# Autodesk Inventor assembly: KZBN17-113-P14-LA25-TC4-TB4-KB21-HB50-ZA3-HA18-AA120
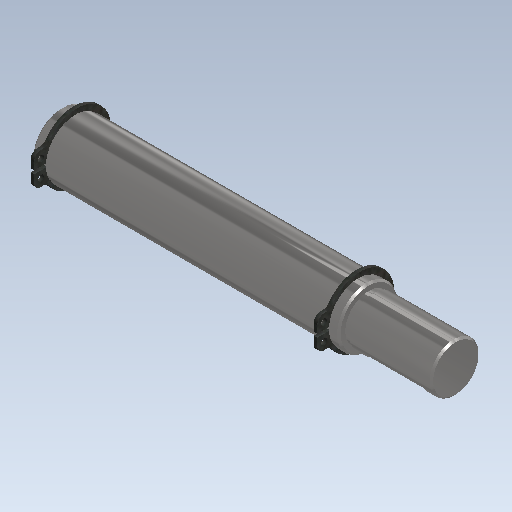
[picture p0: Inventor's stored thumbnail of the model, 512x512]
Saved by Autodesk Inventor 2021.3 (Build 253353000, 353)
## iProperties
Part Number: KZBN17-113-P14-LA25-TC4-TB4-KB21-HB50-ZA3-HA18-AA120
Catalog Web Link: www.cadenas.de
Description: KZBE, KZBN, KZBC, KZBP, KZBF-Driving Shaft - One End Stepped -
Vendor: MISUMI
Document SubType Name: Assembly
Designer: partserver
Manufacturer: MISUMI
Mass: 22.9238 g
Surface Area: 74.0466 cm^2
Volume: 22.9238 cm^3
Density: 1 g/cm^3
Category: PARTsolutions
Company: MISUMI
PSOL_IDENT_0: {$CADENAS_DATA\23d-libs\misumi\metric\11_rotary_shafts\kzbc_asmtab.prj},748 {VTYP=3D},{STYP=ASSTAB},
PSOL_IDENT_1: {NB=KZBN17-113-P14-LA25-TC4-TB4-KB21-HB50-ZA3-HA18-AA120},{LINA=KZBN17-113-P14-LA25-TC4-TB4-KB21-HB5
PSOL_IDENT_2: 0-ZA3-HA18-AA120},{NN=KZBE, KZBN, KZBC, KZBP, KZBF},{DATE=27.07.2021 05:05:24},{GEOMDATE=01.11.2019
PSOL_IDENT_3: 08:16:05},{VERSION=},{LINEID=60},{WBVAR=TS,HARD,ST,L,P,LA,ALT1,MA,MSA,MMA,ALT4,MD,MSD,MMD,ALT2,MB,MS
PSOL_IDENT_4: B,MMB,ALT5,NA,NBALT5,ALT7,TA,ALT6,TC,TB,ALT9,KA,HAALT9,ALT10,KB,HBALT10,KC,HCALT10,ALT12,ZA,HAALT12,
PSOL_IDENT_5: AAALT12,ALT13,ZB,HBALT13,ABALT13,ZC,HCALT13,ACALT13,ALT15,SA,ALT16,SC,ALT18,WA,GA,AAALT18,ALT19,WB,G
PSOL_IDENT_6: B,ABALT19,WC,GC,ACALT19},{WBNUMERIC=L,P,LA,MA,MSA,MMA,MD,MSD,MMD,MB,MSB,MMB,TA,TC,TB,KA,HAALT9,KB,HB
PSOL_IDENT_7: ALT10,KC,HCALT10,ZA,HAALT12,AAALT12,ZB,HBALT13,ABALT13,ZC,HCALT13,ACALT13,SA,SC,WA,GA,AAALT18,WB,GB,
PSOL_IDENT_8: ABALT19,WC,GC,ACALT19}  {NB=KZBN17-113-P14-LA25-TC4-TB4-KB21-HB50-ZA3-HA18-AA120},{LINA=KZBN17-113-P
PSOL_IDENT_9: 14-LA25-TC4-TB4-KB21-HB50-ZA3-HA18-AA120},{KT=DUMMY},{PN=KZBN17-113-P14-LA25-TC4-TB4-KB21-HB50-ZA3-H
PSOL_IDENT_10: A18-AA120},{TYPE=KZBN},{D=17},{TS=h6},{TSALG= 'h7','h7','h6','h6' },{HARD=-},{HARDALG= '-','-','IHSH
PSOL_IDENT_11: 50','Induction Hardened Surface Hardness 50HRC' },{ST=-},{STALG= '-','-','BO','Black Oxide','ENP','E
PSOL_IDENT_12: lectroless Nickel Plating'},{L=113.0},{LALG=[100:400/0.5]},{P=14},{PALG=[10:16/1]},{PMIN=10},{PMAX=1
PSOL_IDENT_13: 6},{LA=25.0},{LAALG=[10:56.5/0.5]},{LAMIN=10.0},{LAMAX=56.5},{CIFCC=0.5},{CIFR=0.0},{ALT1=},{ALT1ALG=
PSOL_IDENT_14: '','Not applicable' },{ALT1PN=},{MA=0},{MAALG=[0]},{MAMIN=0},{MAMAX=0},{MSA=0},{MSAALG=[0]},{MSAMIN=
PSOL_IDENT_15: 0},{MSAMAX=0},{MMA=0},{MMAALG=[0]},{MMAMIN=0},{MMAMAX=0},{MALT1=0},{APITCH=0.00},{ALT4=},{ALT4ALG= ''
PSOL_IDENT_16: ,'w/o Shaft End D Threaded Left End','MSD','with MSD (Fine (Standard) JIS 6h (Class 2))','MMD','with
PSOL_IDENT_17: MMD (Fine (Precision) JIS 4h (Class 1))' },{ALT4PN=},{MD=0},{MDALG=[0]},{MDMIN=0},{MDMAX=0},{MSD=0}
PSOL_IDENT_18: ,{MSDALG=[0]},{MSDMIN=0},{MSDMAX=0},{MMD=0},{MMDALG=[0]},{MMDMIN=0},{MMDMAX=0},{MALT4=0},{DPITCH=0.0
PSOL_IDENT_19: 0},{MDPITCH=0},{MSDPITCH=1},{ALT2=},{ALT2ALG= '','w/o Shaft End D Threaded Right End','MSB','with MS
PSOL_IDENT_20: B (Fine (Standard) JIS 6h (Class 2))','MMB','with MMB (Fine (Precision) JIS 4h (Class 1))' },{ALT2PN=
PSOL_IDENT_21: },{MB=0},{MBALG=[0]},{MBMIN=0},{MBMAX=0},{MSB=0},{MSBALG=[0]},{MSBMIN=0},{MSBMAX=0},{MMB=0},{MMBALG=
PSOL_IDENT_22: [0]},{MMBMIN=0},{MMBMAX=0},{MALT2=0},{BPITCH=0.00},{ALT5=},{ALT5ALG= '','w/o Tapped Ends','NA','with
PSOL_IDENT_23: NA (Tapped Left End)','NB','with NB (Tapped Right End)','NANB','with NA + NB (Tapped Both Ends)' },
PSOL_IDENT_24: {ALT5PN=},{NA=0},{NAALG= '0','N/A' },{NAMAX=10},{NA1=0},{NAL=0},{PITCHA=0},{NBALT5=0},{NBALT5ALG= '0'
PSOL_IDENT_25: ,'N/A' },{NBMAX=12},{NBMAX1=24},{NBMAX2=12},{NBMAX3=12},{NBMAX4=0},{NB1=0},{NBL=0},{PITCHB=0},{CIFNA=
PSOL_IDENT_26: 0},{ALT7=},{ALT7ALG=  '','w/o Shaft End P Retaining Ring Groove','TA','with TA (Shaft End P Retainin
PSOL_IDENT_27: g Ring Groove)' },{ALT7PN=},{TA=0},{TAALG=[0]},{TAMIN=4},{TAMAX=22},{DDALT7=0.0},{MMALT7=0.00},{ALT6=
PSOL_IDENT_28: TCTB},{ALT6ALG=  '','w/o Shaft End D Retaining Ring Grooves','TC','with TC (Shaft End D Retaining Ri
PSOL_IDENT_29: ng Groove Left End)','TB','with TB (Shaft End D Retaining Ring Groove Right End)','TCTB','with TC +
PSOL_IDENT_30: TB (Shaft End D Retaining Ring Grooves Both Ends)' },{ALT6PN=-TC4-TB4},{TC=4},{TCALG=[4:82/1]},{TCMI
PSOL_IDENT_31: N=4},{TCMAX=82},{TB=4},{TBALG=[4:86/1]},{TBMIN=4},{TBMAX=86},{DDALT6=16.2},{MMALT6=1.15},{ALT9=},{AL
PSOL_IDENT_32: T9ALG= '','w/o Shaft End P Key Groove','KA','with KA (Shaft End P Key Groove)' },{ALT9PN=},{KA=0},{K
PSOL_IDENT_33: AALG=[0]},{KAMIN=0},{KAMAX=18},{HAALT9=0},{HAALT9ALG=[0]},{HAALT9MIN=5},{HAALT9MAX=23},{PBB=5},{PTT=
PSOL_IDENT_34: 3.0},{ALT10=KB},{ALT10ALG= '','w/o Shaft End D Key Grooves','KB','with KB (Shaft End D Key Groove)','
PSOL_IDENT_35: KBKC','with KB + KC (Shaft End D Two Key Grooves)' },{ALT10PN=-KB21-HB50},{KB=21},{KBALG=[2:83/1]},{
PSOL_IDENT_36: KBMIN=2},{KBMAX1=83},{KBMAX2=76},{HBALT10=50},{HBALT10ALG=[5:67/1]},{HBALT10MIN=5},{HBALT10MAX1=67},
PSOL_IDENT_37: {HBALT10MAX2=60},{KC=0},{KCALG=[0]},{KCMIN=73},{KCMAX=83},{HCALT10=0},{HCALT10ALG=[0]},{HCALT10MIN=5
PSOL_IDENT_38: },{HCALT10MAX=88},{DBB=5},{DTT=3.0},{ALT12=ZA},{ALT12ALG= '','w/o Shaft End P Key Groove + Set Screw
PSOL_IDENT_39: Flat','ZA','with ZA (Shaft End P Key Groove + Set Screw Flat)' },{ALT12PN=-ZA3-HA18-AA120},{ZA=3},{
PSOL_IDENT_40: ZAALG=[0:18/1]},{ZAMIN=0},{ZAMAX=18},{HAALT12=18},{HAALT12ALG=[5:20/1]},{HAALT12MIN=5},{HAALT12MAX=2
PSOL_IDENT_41: 0},{AAALT12=120},{AAALT12ALG=[60:300/30]},{PH=1},{ALT13=},{ALT13ALG= '','Not applicable' },{ALT13PN=
PSOL_IDENT_42: },{ZB=0},{ZBALG=[0]},{ZBMIN=2},{ZBMAX1=83},{ZBMAX2=76},{HBALT13=0},{HBALT13ALG=[0]},{HBALT13MIN=5},{
PSOL_IDENT_43: HBALT13MAX1=88},{HBALT13MAX2=81},{ABALT13=0},{ABALT13ALG=[0]},{ZC=0},{ZCALG=[0]},{ZCMIN=2},{ZCMAX=83
PSOL_IDENT_44: },{HCALT13=0},{HCALT13ALG=[0]},{HCALT13MIN=5},{HCALT13MAX=88},{ACALT13=0},{ACALT13ALG=[0]},{DH=0},{A
PSOL_IDENT_45: LT15=},{ALT15ALG= '', 'w/o Shaft End P Wrench Flats', 'SA', 'with SA (Shaft End P Wrench Flats)' },{
PSOL_IDENT_46: ALT15PN=},{SA=0},{SAALG=[0]},{SAMIN=0},{SAMAX=25},{WALT15=0.0},{LLALT15=0},{ALT16=},{ALT16ALG= '', '
PSOL_IDENT_47: w/o Shaft End D Wrench Flats', 'SC', 'with SC (Shaft End D Wrench Flats)' },{ALT16PN=},{SC=0},{SCALG=
PSOL_IDENT_48: [0]},{SCMIN=2},{SCMAX=88},{WALT16=0},{LLALT16=0},{ALT18=},{ALT18ALG= '','Not applicable' },{ALT18PN=
PSOL_IDENT_49: },{WA=0},{WAALG=[0]},{WAMIN=0},{WAMAX=22},{GA=0},{GAALG=[0]},{GAMIN=3},{GAMAX=25},{AAALT18=0},{AAALT
PSOL_IDENT_50: 18ALG=[0]},{ALT19=},{ALT19ALG= '','w/o Shaft End D 2 Set Screw Flats (Angle Specified)','WB','with W
PSOL_IDENT_51: B (Shaft End D 2 Set Screw Flats (Angle Specified))','WBWC','with WB + WC (Shaft End D Two 2 Set Scr
PSOL_IDENT_52: ew Flats (Angle Specified))' },{ALT19PN=},{WB=0},{WBALG=[0]},{WBMIN=2},{WBMAX1=85},{WBMAX2=80},{GB=0
PSOL_IDENT_53: },{GBALG=[0]},{GBMIN=3},{GBMAX1=88},{GBMAX2=83},{ABALT19=0},{ABALT19ALG=[0]},{WC=0},{WCALG=[0]},{WCM
PSOL_IDENT_54: IN=2},{WCMAX=85},{GC=0},{GCALG=[0]},{GCMIN=3},{GCMAX=88},{ACALT19=0},{ACALT19ALG=[0]},{ERRORPN=},{ER
PSOL_IDENT_55: RORPALT16=OK},{ERRORPALT19=OK},{ERRORALT15=OK},{ERRORALT17=OK},{ERRORALT115=OK},{ERRORALT118=OK},{ER
PSOL_IDENT_56: RORALT25=OK},{ERRORALT26=OK},{ERRORALT216=OK},{ERRORALT219=OK},{ERRORALT45=OK},{ERRORALT46=OK},{ERRO
PSOL_IDENT_57: RALT416=OK},{ERRORALT419=OK},{ERRORALT59=OK},{ERRORALT510=OK},{ERRORALT512=OK},{ERRORALT513=OK},{ERR
PSOL_IDENT_58: ORALT515=OK},{ERRORALT516=OK},{ERRORALT518=OK},{ERRORALT519=OK},{ERRORALT610=OK},{ERRORALT613=OK},{E
PSOL_IDENT_59: RRORALT616=OK},{ERRORALT619=OK},{ERRORALT79=OK},{ERRORALT712=OK},{ERRORALT715=OK},{ERRORALT718=OK},{
PSOL_IDENT_60: ERRORALT915=OK},{ERRORALT918=OK},{ERRORALT1016=OK},{ERRORALT1019=OK},{ERRORALT1215=OK},{ERRORALT1316=
PSOL_IDENT_61: OK},{ERRORALT1518=OK},{ERRORALT1619=OK},{PPATH=11_components/kzbc/kzbc_asmtpl.prj}
NB: KZBN17-113-P14-LA25-TC4-TB4-KB21-HB50-ZA3-HA18-AA120
NN: KZBE, KZBN, KZBC, KZBP, KZBF
NT: Driving Shaft - One End Stepped -
NBSYN: $PN.
LINA: KZBN17-113-P14-LA25-TC4-TB4-KB21-HB50-ZA3-HA18-AA120
CATALOG: Misumi
PN: KZBN17-113-P14-LA25-TC4-TB4-KB21-HB50-ZA3-HA18-AA120
D: 17
TS: h6
HARD: -
ST: -
L: 113
P: 14
LA: 25
ALT1: Not applicable
MA: 0
MSA: 0
MMA: 0
ALT4: w/o Shaft End D Threaded Left End
MD: 0
MSD: 0
MMD: 0
ALT2: w/o Shaft End D Threaded Right End
MB: 0
MSB: 0
MMB: 0
ALT5: w/o Tapped Ends
NA: N/A
NBALT5: N/A
ALT7: w/o Shaft End P Retaining Ring Groove
TA: 0
DDALT7: 0
MMALT7: 0
ALT6: with TC + TB (Shaft End D Retaining Ring Grooves Both Ends)
TC: 4
TB: 4
DDALT6: 16.2
MMALT6: 1.15
ALT9: w/o Shaft End P Key Groove
KA: 0
HAALT9: 0
ALT10: with KB (Shaft End D Key Groove)
KB: 21
HBALT10: 50
KC: 0
HCALT10: 0
ALT12: with ZA (Shaft End P Key Groove + Set Screw Flat)
ZA: 3
HAALT12: 18
AAALT12: 120
PH: 1
ALT13: Not applicable
ZB: 0
HBALT13: 0
ABALT13: 0
ZC: 0
HCALT13: 0
ACALT13: 0
DH: 0
ALT15: w/o Shaft End P Wrench Flats
SA: 0
WALT15: 0
LLALT15: 0
ALT16: w/o Shaft End D Wrench Flats
SC: 0
WALT16: 0
LLALT16: 0
ALT18: Not applicable
WA: 0
GA: 0
AAALT18: 0
ALT19: w/o Shaft End D 2 Set Screw Flats (Angle Specified)
WB: 0
GB: 0
ABALT19: 0
WC: 0
GC: 0
ACALT19: 0
SUPPLIER: MISUMI
ARTICLENO: KZBN17-113-P14-LA25-TC4-TB4-KB21-HB50-ZA3-HA18-AA120
BOMINFO: KZBN17-113-P14-LA25-TC4-TB4-KB21-HB50-ZA3-HA18-AA120
CREATOR: CADENAS GmbH
Title: KZBN17-113-P14-LA25-TC4-TB4-KB21-HB50-ZA3-HA18-AA120
Author: Cadenas PARTsolutions
Comments: Driving Shaft - One End Stepped -
## Documents named in this file (3)
- C:\Users\nxf77172\Desktop\mechanical_cleaned\custom_parts\drivetrain\wheel_axle\AIS2020\KZBN17-113-P14-LA25-TC4-TB4-KB21-HB50-ZA3-HA18-AA120.iam
- C:\Users\nxf77172\Desktop\mechanical_cleaned\custom_parts\drivetrain\wheel_axle\AIS2020\KZBN17-113-P14-LA25-TC4-TB4-KB21-HB50-ZA3-HA18-AA120_b.ipt
- C:\Users\nxf77172\Desktop\mechanical_cleaned\custom_parts\drivetrain\wheel_axle\AIS2020\RRING-C-EXT-17.ipt
## Components (3 placed, 2 different names)
1. KZBN17-113-P14-LA25-TC4-TB4-KB21-HB50-ZA3-HA18-AA120_b:1 — to_c_ring_2_XY@1 <-> 1_XY@2, to_c_ring_2_Z@1 <-> 1_Z@2, to_c_ring_2_YZ@1 <-> 1_YZ@2, to_c_ring_3_XY@1 <-> 1_XY@3, to_c_ring_3_Z@1 <-> 1_Z@3, to_c_ring_3_YZ@1 <-> 1_YZ@3
2. RRING-C-EXT-17:1 — to_c_ring_2_XY@1 <-> 1_XY@2, to_c_ring_2_Z@1 <-> 1_Z@2, to_c_ring_2_YZ@1 <-> 1_YZ@2
3. RRING-C-EXT-17:2 — to_c_ring_3_XY@1 <-> 1_XY@3, to_c_ring_3_Z@1 <-> 1_Z@3, to_c_ring_3_YZ@1 <-> 1_YZ@3
## Relationships (6: Mate 4, Angle 2)
- to_c_ring_2_XY@1 <-> 1_XY@2 [Mate]: KZBN17-113-P14-LA25-TC4-TB4-KB21-HB50-ZA3-HA18-AA120_b:1 ↔ RRING-C-EXT-17:1
- to_c_ring_2_Z@1 <-> 1_Z@2 [Mate]: KZBN17-113-P14-LA25-TC4-TB4-KB21-HB50-ZA3-HA18-AA120_b:1 ↔ RRING-C-EXT-17:1
- to_c_ring_2_YZ@1 <-> 1_YZ@2 [Angle] (0 deg): KZBN17-113-P14-LA25-TC4-TB4-KB21-HB50-ZA3-HA18-AA120_b:1 ↔ RRING-C-EXT-17:1
- to_c_ring_3_XY@1 <-> 1_XY@3 [Mate]: KZBN17-113-P14-LA25-TC4-TB4-KB21-HB50-ZA3-HA18-AA120_b:1 ↔ RRING-C-EXT-17:2
- to_c_ring_3_Z@1 <-> 1_Z@3 [Mate]: KZBN17-113-P14-LA25-TC4-TB4-KB21-HB50-ZA3-HA18-AA120_b:1 ↔ RRING-C-EXT-17:2
- to_c_ring_3_YZ@1 <-> 1_YZ@3 [Angle] (0 deg): KZBN17-113-P14-LA25-TC4-TB4-KB21-HB50-ZA3-HA18-AA120_b:1 ↔ RRING-C-EXT-17:2
